# Autodesk Inventor assembly: Revised_Tilt
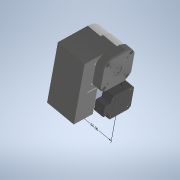
[picture p0: Inventor's stored thumbnail of the model, 180x180]
Saved by Autodesk Inventor 2022 (Build 260153000, 153)
## iProperties
Created: 2022-02-21
Part Number: Revised_Tilt
Document SubType Name: Assembly
Designer: Mlees
Author: Mlees
## Documents named in this file (13)
- C:\Users\Mlees\Desktop\504Engineering\Stepper-Servo_Based_Robotic_Arm\Designs\Version_7\Revised_Tilt.iam
- C:\Users\Mlees\Desktop\504Engineering\Stepper-Servo_Based_Robotic_Arm\Designs\Version_7\Created_Parts\Combined_Gear_Box_Modified_2.ipt
- C:\Users\Mlees\Desktop\504Engineering\Stepper-Servo_Based_Robotic_Arm\Designs\Version_7\Created_Parts\Combined_Gear_Box_Modified_3.ipt
- C:\Users\Mlees\Desktop\504Engineering\Stepper-Servo_Based_Robotic_Arm\Designs\Version_7\Downloaded_Parts\124125202-9-stp-mtr-17040w\stp-mtr-17040w.ipt
- C:\Users\Mlees\Desktop\504Engineering\Stepper-Servo_Based_Robotic_Arm\Designs\Version_7\Created_Parts\Gear_Cover_modified.ipt
- C:\Users\Mlees\Desktop\504Engineering\Stepper-Servo_Based_Robotic_Arm\Designs\Version_7\Downloaded_Parts\9403T15_Tight-Tolerance High-Strength 7075 Aluminum Rod.ipt
- C:\Users\Mlees\Desktop\504Engineering\Stepper-Servo_Based_Robotic_Arm\Designs\Version_7\Downloaded_Parts\GT2 20T Drive Pulley.ipt
- C:\Users\Mlees\Desktop\504Engineering\Stepper-Servo_Based_Robotic_Arm\Designs\Version_7\Downloaded_Parts\GT2 60T Drive Pulley.ipt
- C:\Users\Mlees\Desktop\504Engineering\Stepper-Servo_Based_Robotic_Arm\Designs\Version_7\Created_Parts\24_Teeth_Sun_Gear.ipt
- C:\Users\Mlees\Desktop\504Engineering\Stepper-Servo_Based_Robotic_Arm\Designs\Version_7\Created_Parts\36_Teeth_Planet_Gear.ipt
- C:\Users\Mlees\Desktop\504Engineering\Stepper-Servo_Based_Robotic_Arm\Designs\Version_7\Created_Parts\Planet_Carrier_Modifed_with_sun_gear.ipt
- C:\Users\Mlees\Desktop\504Engineering\Stepper-Servo_Based_Robotic_Arm\Designs\Version_7\Created_Parts\Plamet_Carrier.ipt
- C:\Users\Mlees\Desktop\504Engineering\Stepper-Servo_Based_Robotic_Arm\Designs\Version_7\Downloaded_Parts\91290A113_Black-Oxide Alloy Steel Socket Head Screw.ipt
## Components (22 placed, 12 different names)
1. Combined_Gear_Box_Modified_2:1 — Rigid:1, Rigid:3, Rotational:20
2. Combined_Gear_Box_Modified_3:1 — Rigid:1, Rigid:2
3. stp-mtr-17040w:1 — Rigid:2, Rotational:1
4. Gear_Cover_modified:1 — Rigid:3
5. 9403T15_Tight-Tolerance High-Strength 7075 Aluminum Rod:2 — Rigid:4, Rotational:19
6. GT2 20T Drive Pulley:1 — Rotational:1
7. GT2 60T Drive Pulley:1 — Rotational:19, Rotational:20
8. 24_Teeth_Sun_Gear:1 — Rigid:4, Rigid:5
9. 36_Teeth_Planet_Gear:1 — Rotational:4, Rotational:9
10. 36_Teeth_Planet_Gear:2 — Rotational:5, Rotational:8
11. 36_Teeth_Planet_Gear:3 — Rotational:6, Rotational:7
12. 36_Teeth_Planet_Gear:4 — Rotational:14, Rotational:17
13. 36_Teeth_Planet_Gear:5 — Rotational:13, Rotational:16
14. 36_Teeth_Planet_Gear:6 — Rotational:12, Rotational:15
15. Planet_Carrier_Modifed_with_sun_gear:1 — Rotational:4, Rotational:5, Rotational:6, Rotational:18, Rigid:5
16. Plamet_Carrier:1 — Rotational:12, Rotational:13, Rotational:14, Rotational:18
17. 91290A113_Black-Oxide Alloy Steel Socket Head Screw:1 — Rotational:17
18. 91290A113_Black-Oxide Alloy Steel Socket Head Screw:2 — Rotational:7
19. 91290A113_Black-Oxide Alloy Steel Socket Head Screw:3 — Rotational:15
20. 91290A113_Black-Oxide Alloy Steel Socket Head Screw:4 — Rotational:16
21. 91290A113_Black-Oxide Alloy Steel Socket Head Screw:5 — Rotational:9
22. 91290A113_Black-Oxide Alloy Steel Socket Head Screw:6 — Rotational:8
## Relationships (21: RevoluteJoint 16, WeldJoint 5)
- Rigid:1 [WeldJoint]: Combined_Gear_Box_Modified_2:1 ↔ Combined_Gear_Box_Modified_3:1
- Rigid:2 [WeldJoint]: Combined_Gear_Box_Modified_3:1 ↔ stp-mtr-17040w:1
- Rigid:3 [WeldJoint]: Combined_Gear_Box_Modified_2:1 ↔ Gear_Cover_modified:1
- Rotational:1 [RevoluteJoint] (-5 mm): stp-mtr-17040w:1 ↔ GT2 20T Drive Pulley:1
- Rotational:4 [RevoluteJoint]: 36_Teeth_Planet_Gear:1 ↔ Planet_Carrier_Modifed_with_sun_gear:1
- Rotational:5 [RevoluteJoint]: 36_Teeth_Planet_Gear:2 ↔ Planet_Carrier_Modifed_with_sun_gear:1
- Rotational:6 [RevoluteJoint]: 36_Teeth_Planet_Gear:3 ↔ Planet_Carrier_Modifed_with_sun_gear:1
- Rotational:7 [RevoluteJoint]: 36_Teeth_Planet_Gear:3 ↔ 91290A113_Black-Oxide Alloy Steel Socket Head Screw:2
- Rotational:8 [RevoluteJoint]: 36_Teeth_Planet_Gear:2 ↔ 91290A113_Black-Oxide Alloy Steel Socket Head Screw:6
- Rotational:9 [RevoluteJoint]: 36_Teeth_Planet_Gear:1 ↔ 91290A113_Black-Oxide Alloy Steel Socket Head Screw:5
- Rotational:12 [RevoluteJoint]: 36_Teeth_Planet_Gear:6 ↔ Plamet_Carrier:1
- Rotational:13 [RevoluteJoint]: 36_Teeth_Planet_Gear:5 ↔ Plamet_Carrier:1
- Rotational:14 [RevoluteJoint]: 36_Teeth_Planet_Gear:4 ↔ Plamet_Carrier:1
- Rotational:15 [RevoluteJoint]: 36_Teeth_Planet_Gear:6 ↔ 91290A113_Black-Oxide Alloy Steel Socket Head Screw:3
- Rotational:16 [RevoluteJoint]: 36_Teeth_Planet_Gear:5 ↔ 91290A113_Black-Oxide Alloy Steel Socket Head Screw:4
- Rotational:17 [RevoluteJoint]: 36_Teeth_Planet_Gear:4 ↔ 91290A113_Black-Oxide Alloy Steel Socket Head Screw:1
- Rotational:18 [RevoluteJoint]: Planet_Carrier_Modifed_with_sun_gear:1 ↔ Plamet_Carrier:1
- Rigid:4 [WeldJoint]: 9403T15_Tight-Tolerance High-Strength 7075 Aluminum Rod:2 ↔ 24_Teeth_Sun_Gear:1
- Rotational:19 [RevoluteJoint]: 9403T15_Tight-Tolerance High-Strength 7075 Aluminum Rod:2 ↔ GT2 60T Drive Pulley:1
- Rotational:20 [RevoluteJoint]: Combined_Gear_Box_Modified_2:1 ↔ GT2 60T Drive Pulley:1
- Rigid:5 [WeldJoint]: 24_Teeth_Sun_Gear:1 ↔ Planet_Carrier_Modifed_with_sun_gear:1
